# Autodesk Inventor assembly: sumoltaneous-equations
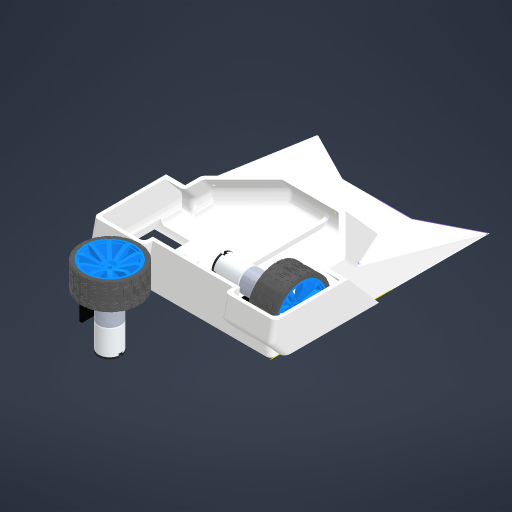
[picture p0: Inventor's stored thumbnail of the model, 512x512]
Saved by Autodesk Inventor 2023 (Build 270158000, 158)
## iProperties
Created: 2022-06-23
Part Number: sumoltaneous-equations
Document SubType Name: Assembly
Designer: Dan
Author: Dan
## Documents named in this file (3)
- C:\Users\x43dn\Desktop\sumoltaneous-equations\sumoltaneous-equations-inventor\sumoltaneous-equations.iam
- C:\Users\x43dn\Desktop\sumoltaneous-equations\sumoltaneous-equations-inventor\chassis.ipt
- C:\Users\x43dn\Desktop\sumoltaneous-equations\sumoltaneous-equations-inventor\wheel.iam
## Components (3 placed, 2 different names)
1. chassis:1 — Mate:1, Mate:2
2. wheel:1 [sub-assembly]
3. wheel:2 [sub-assembly] — Mate:1, Mate:2
## Relationships (2: Mate 2)
- Mate:1: chassis:1 ↔ wheel:2
- Mate:2: chassis:1 ↔ wheel:2
